# Autodesk Inventor assembly: CC2x2
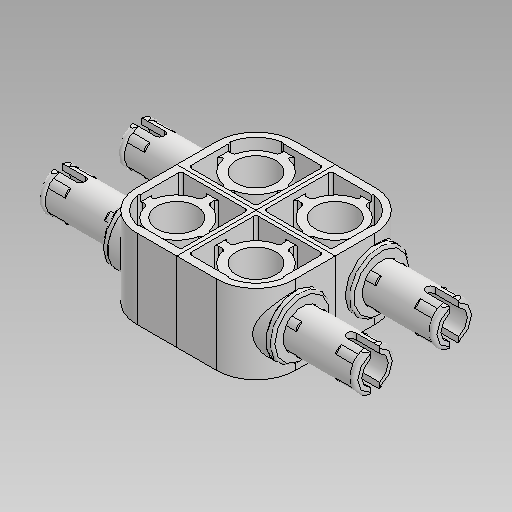
[picture p0: Inventor's stored thumbnail of the model, 512x512]
Saved by Autodesk Inventor 2020 (Build 240168000, 168)
## iProperties
Created: 2019-05-05
Part Number: CC2x2
Document SubType Name: Assembly
Designer: Varga Daniel
Author: Varga Daniel
## Documents named in this file (4)
- C:\!_Dani\!_cloud\OneDrive\!_munka\Revolution\StructuralParts\Connector Boxes\Connector Cubes\CC2x2.iam
- C:\!_Dani\!_cloud\OneDrive\!_munka\Revolution\StructuralParts\Connector Boxes\Connector_box_corner.ipt
- C:\!_Dani\!_cloud\OneDrive\!_munka\Revolution\StructuralParts\Connector pins\CP1_base\CP1_base-one_side_anti_skid.ipt
- C:\!_Dani\!_cloud\OneDrive\!_munka\Revolution\StructuralParts\Connector pins\CP1_base.ipt
## Components (8 placed, 2 different names)
1. Connector_box_corner:1 — Mate:1, Mate:2, Flush:1, Flush:2, Flush:3, Flush:4, Flush:5, Mate:5, Mate:8, Flush:7
2. Connector_box_corner:2 — Mate:1, Mate:3, Flush:1, Flush:5, Flush:6, Mate:4, Mate:10, Flush:9
3. Connector_box_corner:3 — Mate:2, Flush:3, Flush:4, Mate:7, Flush:8, Mate:9
4. Connector_box_corner:4 — Mate:3, Flush:2, Flush:6, Mate:6, Mate:11, Flush:10
5. CP1_base-one_side_anti_skid:1 — Mate:6, Mate:11, Flush:10
6. CP1_base-one_side_anti_skid:2 — Mate:5, Mate:8, Flush:7
7. CP1_base-one_side_anti_skid:3 — Mate:4, Mate:10, Flush:9
8. CP1_base-one_side_anti_skid:4 — Mate:7, Flush:8, Mate:9
## Relationships (21: Mate 11, Flush 10)
- Mate:1: Connector_box_corner:1 ↔ Connector_box_corner:2
- Mate:2: Connector_box_corner:1 ↔ Connector_box_corner:3
- Mate:3: Connector_box_corner:2 ↔ Connector_box_corner:4
- Flush:1: Connector_box_corner:1 ↔ Connector_box_corner:2
- Flush:2: Connector_box_corner:1 ↔ Connector_box_corner:4
- Flush:3: Connector_box_corner:1 ↔ Connector_box_corner:3
- Flush:4: Connector_box_corner:1 ↔ Connector_box_corner:3
- Flush:5: Connector_box_corner:1 ↔ Connector_box_corner:2
- Flush:6: Connector_box_corner:2 ↔ Connector_box_corner:4
- Mate:4: Connector_box_corner:2 ↔ CP1_base-one_side_anti_skid:3
- Mate:5: Connector_box_corner:1 ↔ CP1_base-one_side_anti_skid:2
- Mate:6: Connector_box_corner:4 ↔ CP1_base-one_side_anti_skid:1
- Mate:7: Connector_box_corner:3 ↔ CP1_base-one_side_anti_skid:4
- Mate:8: Connector_box_corner:1 ↔ CP1_base-one_side_anti_skid:2
- Flush:7: Connector_box_corner:1 ↔ CP1_base-one_side_anti_skid:2
- Flush:8: Connector_box_corner:3 ↔ CP1_base-one_side_anti_skid:4
- Mate:9: Connector_box_corner:3 ↔ CP1_base-one_side_anti_skid:4
- Mate:10: Connector_box_corner:2 ↔ CP1_base-one_side_anti_skid:3
- Flush:9: Connector_box_corner:2 ↔ CP1_base-one_side_anti_skid:3
- Mate:11: Connector_box_corner:4 ↔ CP1_base-one_side_anti_skid:1
- Flush:10: Connector_box_corner:4 ↔ CP1_base-one_side_anti_skid:1
